# Autodesk Inventor assembly: Cartridge Clamp1771613
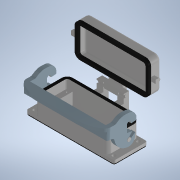
[picture p0: Inventor's stored thumbnail of the model, 180x180]
Saved by Autodesk Inventor 2021 (Build 250183000, 183)
## iProperties
Created: 2008-08-08
Part Number: Cartridge Clamp1771613
Description: SolidDesigner STEP Export
Document SubType Name: Assembly
Designer: jgray
Title: 1771613.stp
## Documents named in this file (2)
- M:\Printed Electronics\Gas Sensors\Prototypes\Prototype II - Cartridge Reader\Full Cart Interface V3 28-5-20\Workspaces\Workspace\Workspaces\Workspace\Externally supplied Parts\Cartridge Clamp1771613.iam
- M:\Printed Electronics\Gas Sensors\Prototypes\Prototype II - Cartridge Reader\Full Cart Interface V3 28-5-20\Workspaces\Workspace\Workspaces\Workspace\Externally supplied Parts\Cartridge Clamp1771613.ipt
## Components (1 placed, 1 different names)
1. 1 — Mate:1, Mate:2, Mate:3
## Relationships (3: Mate 3)
- Mate:1: 1
- Mate:2: 1
- Mate:3: 1
